# Autodesk Inventor assembly: PS20023
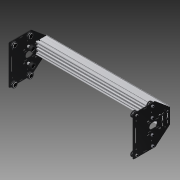
[picture p0: Inventor's stored thumbnail of the model, 180x180]
Saved by Autodesk Inventor 2014 (Build 180170000, 170)
## iProperties
Created: 2013-09-18
Part Number: PS20023
Document SubType Name: Assembly
Designer: Edward
Author: Edward
## Documents named in this file (6)
- C:\Users\Edward\Documents\GitHub\Shapeoko_2\Autodesk_Inventor_Project\PS20023.iam
- C:\Users\Edward\Documents\GitHub\Shapeoko_2\Autodesk_Inventor_Project\PS20022.iam
- C:\Users\Edward\Documents\GitHub\Shapeoko_2\Autodesk_Inventor_Project\PS20020.iam
- C:\Users\Edward\Documents\GitHub\Shapeoko_2\Autodesk_Inventor_Project\25286-02.ipt
- C:\Users\Edward\Documents\GitHub\Shapeoko_2\Autodesk_Inventor_Project\25287-02.ipt
- C:\Users\Edward\Documents\GitHub\Shapeoko_2\Autodesk_Inventor_Project\PS20008.ipt
## Components (22 placed, 5 different names)
1. PS20008:1 — Flush:6, Flush:7
2. PS20022:1 [sub-assembly] — Flush:6
3. PS20022:2 [sub-assembly] — Mate:9
4. PS20020:1 [sub-assembly]
5. PS20020:2 [sub-assembly]
6. 25286-02:1
7. 25287-02:1
8. 25286-02:2
9. 25287-02:2
10. 25286-02:3
11. 25287-02:3
12. 25286-02:4
13. 25287-02:4
14. PS20008:2 — Mate:9, Flush:7, Insert:11, Insert:13, Insert:16, Insert:17
15. 25286-02:5
16. 25287-02:5 — Insert:11
17. 25286-02:6
18. 25287-02:6 — Insert:13
19. 25286-02:7
20. 25287-02:7 — Insert:17
21. 25286-02:8
22. 25287-02:8 — Insert:16
## Relationships (31: Insert 17, Mate 8, Flush 6)
- [Flush]: PS20022:1 ↔ PS20022:2
- [Mate] (500 mm): PS20022:1 ↔ PS20022:2
- [Mate]: PS20008:1 ↔ PS20022:1
- [Mate]: PS20008:1 ↔ PS20022:2
- [Flush]: PS20008:1 ↔ PS20022:2
- [Insert]: PS20008:1 ↔ PS20022:2
- [Mate]: PS20008:1 ↔ PS20020:1
- [Flush] (3 mm): PS20008:1 ↔ PS20020:1
- [Mate]: PS20022:1 ↔ PS20020:1
- [Mate]: PS20008:1 ↔ PS20020:2
- [Flush] (3 mm): PS20008:1 ↔ PS20020:2
- [Mate]: PS20022:2 ↔ PS20020:2
- [Insert]: 25286-02:1 ↔ 25287-02:1
- [Insert]: 25286-02:2 ↔ 25287-02:2
- [Insert] (3.4163 mm): PS20008:1 ↔ 25287-02:1
- [Insert] (3.4163 mm): PS20008:1 ↔ 25287-02:2
- [Insert]: 25286-02:3 ↔ 25287-02:3
- [Insert]: 25286-02:4 ↔ 25287-02:4
- [Insert] (3.4163 mm): PS20008:1 ↔ 25287-02:4
- [Insert] (3.4163 mm): PS20008:1 ↔ 25287-02:3
- Flush:6: PS20008:1 ↔ PS20022:1
- Mate:9: PS20022:2 ↔ PS20008:2
- Flush:7: PS20008:1 ↔ PS20008:2
- [Insert]: 25286-02:5 ↔ 25287-02:5
- Insert:11 (2.36 mm): PS20008:2 ↔ 25287-02:5
- [Insert]: 25286-02:6 ↔ 25287-02:6
- Insert:13 (2.36 mm): PS20008:2 ↔ 25287-02:6
- [Insert]: 25286-02:7 ↔ 25287-02:7
- [Insert]: 25286-02:8 ↔ 25287-02:8
- Insert:16 (2.36 mm): PS20008:2 ↔ 25287-02:8
- Insert:17 (2.36 mm): PS20008:2 ↔ 25287-02:7
## Named parameters: d101_d55_d51 = 0 mm, d102_d55_d51 = 0 mm, d105_d55_d51 = 0 mm, d106_d55_d51 = 0 mm, d26_d101_d55_d51 = 0 mm, d28_d101_d55_d51 = 0 mm, d30_d101_d55_d51 = 0 mm, d31_d101_d55_d51 = 0 mm
